# Autodesk Inventor assembly: Modul
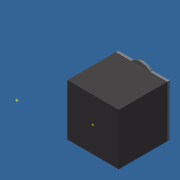
[picture p0: Inventor's stored thumbnail of the model, 180x180]
Saved by Autodesk Inventor 2018.2 (Build 222227000, 227)
## iProperties
Company: Fraunhofer ILT
Created: 2018-10-15
Part Number: Modul
Material: geeigneten Werkstoff auswählen !
Document SubType Name: Assembly
Designer: N.Grubert
Title: =Description
Author: N.Grubert
## Documents named in this file (5)
- C:\Users\GRUBERT\Documents\COSIMA-Laserstar\CAD\Modul.iam
- C:\Users\GRUBERT\Documents\COSIMA-Laserstar\CAD\Modul Deckel.ipt
- C:\Users\GRUBERT\Documents\COSIMA-Laserstar\CAD\Modul Gehäuse.ipt
- C:\Users\GRUBERT\Documents\COSIMA-Laserstar\CAD\SlavesSammelplatine.iam
- C:\Users\GRUBERT\Documents\COSIMA-Laserstar\CAD\Photodiodendummie.ipt
## Components (7 placed, 4 different names)
1. Modul Deckel:1 — Passend:1, Fluchtend:1, Fluchtend:2, Passend:12, Passend:13, Winkel:1, Fluchtend:9
2. Modul Gehäuse:1 — Passend:1, Fluchtend:1, Fluchtend:2, Passend:2, Passend:3, Passend:4, Passend:5, Passend:6, Passend:7
3. SlavesSammelplatine:1 [sub-assembly] — Passend:5, Passend:6, Passend:7
4. Photodiodendummie:1 — Fluchtend:3, Passend:8, Fluchtend:4
5. Photodiodendummie:2 — Fluchtend:3, Passend:8, Fluchtend:4, Fluchtend:7, Passend:10, Fluchtend:8, Fluchtend:9
6. Photodiodendummie:3 — Fluchtend:5, Passend:9, Fluchtend:6, Fluchtend:7, Passend:10, Fluchtend:8, Passend:13, Winkel:1
7. Photodiodendummie:4 — Fluchtend:5, Passend:9, Fluchtend:6, Passend:12
## Relationships (22: Mate 12, Flush 9, Angle 1)
- Passend:1 [Mate]: Modul Deckel:1 ↔ Modul Gehäuse:1
- Fluchtend:1 [Flush]: Modul Deckel:1 ↔ Modul Gehäuse:1
- Fluchtend:2 [Flush]: Modul Deckel:1 ↔ Modul Gehäuse:1
- Passend:2 [Mate]: Modul Gehäuse:1
- Passend:3 [Mate]: Modul Gehäuse:1
- Passend:4 [Mate]: Modul Gehäuse:1
- Passend:5 [Mate] (5 mm): Modul Gehäuse:1 ↔ SlavesSammelplatine:1
- Passend:6 [Mate] (16.25 mm): Modul Gehäuse:1 ↔ SlavesSammelplatine:1
- Passend:7 [Mate]: Modul Gehäuse:1 ↔ SlavesSammelplatine:1
- Fluchtend:3 [Flush]: Photodiodendummie:1 ↔ Photodiodendummie:2
- Passend:8 [Mate] (25 mm): Photodiodendummie:1 ↔ Photodiodendummie:2
- Fluchtend:4 [Flush]: Photodiodendummie:1 ↔ Photodiodendummie:2
- Fluchtend:5 [Flush]: Photodiodendummie:3 ↔ Photodiodendummie:4
- Passend:9 [Mate] (25 mm): Photodiodendummie:3 ↔ Photodiodendummie:4
- Fluchtend:6 [Flush]: Photodiodendummie:3 ↔ Photodiodendummie:4
- Fluchtend:7 [Flush]: Photodiodendummie:2 ↔ Photodiodendummie:3
- Passend:10 [Mate] (25 mm): Photodiodendummie:2 ↔ Photodiodendummie:3
- Fluchtend:8 [Flush]: Photodiodendummie:2 ↔ Photodiodendummie:3
- Passend:12 [Mate] (17.6777 mm): Modul Deckel:1 ↔ Photodiodendummie:4
- Passend:13 [Mate] (17.6777 mm): Modul Deckel:1 ↔ Photodiodendummie:3
- Winkel:1 [Angle] (0 deg): Modul Deckel:1 ↔ Photodiodendummie:3
- Fluchtend:9 [Flush]: Modul Deckel:1 ↔ Photodiodendummie:2
